# Autodesk Inventor assembly: Double door
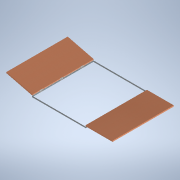
[picture p0: Inventor's stored thumbnail of the model, 180x180]
Saved by Autodesk Inventor 2021 (Build 250183000, 183)
## iProperties
Created: 2021-07-31
Part Number: Double door
Document SubType Name: Assembly
Designer: Shammy Haider
Author: Shammy Haider
## Documents named in this file (4)
- D:\Designing\Autodesk inventor\Wood Door\Double door.iam
- D:\Designing\Autodesk inventor\Wood Door\Frame2.ipt
- D:\Designing\Autodesk inventor\Wood Door\Hinge assembly.iam
- D:\Designing\Autodesk inventor\Wood Door\Door.ipt
## Components (9 placed, 3 different names)
1. Frame2:1 — Mate:1, Mate:2, Mate:3, Mate:4, Mate:5, Mate:6, Mate:7, Mate:8, Mate:9, Mate:10, Mate:11, Mate:12, Mate:13, Mate:14, Mate:15, Mate:16, Mate:17, Mate:18
2. Hinge assembly:1 [sub-assembly] — Mate:1, Mate:2, Mate:3, Mate:20, Mate:23
3. Hinge assembly:2 [sub-assembly] — Mate:13, Mate:16, Mate:17, Mate:21, Mate:22
4. Hinge assembly:3 [sub-assembly] — Mate:14, Mate:15, Mate:18, Mate:19
5. Hinge assembly:4 [sub-assembly] — Mate:10, Mate:11, Mate:12, Mate:26
6. Hinge assembly:5 [sub-assembly] — Mate:7, Mate:8, Mate:9, Mate:25, Mate:27
7. Hinge assembly:6 [sub-assembly] — Mate:4, Mate:5, Mate:6, Mate:24
8. Door:2 — Mate:19, Mate:20, Mate:21, Mate:22, Mate:23
9. Door:3 — Mate:24, Mate:25, Mate:26, Mate:27
## Relationships (27: Mate 27)
- Mate:1: Frame2:1 ↔ Hinge assembly:1
- Mate:2: Frame2:1 ↔ Hinge assembly:1
- Mate:3: Frame2:1 ↔ Hinge assembly:1
- Mate:4: Frame2:1 ↔ Hinge assembly:6
- Mate:5: Frame2:1 ↔ Hinge assembly:6
- Mate:6: Frame2:1 ↔ Hinge assembly:6
- Mate:7: Frame2:1 ↔ Hinge assembly:5
- Mate:8: Frame2:1 ↔ Hinge assembly:5
- Mate:9: Frame2:1 ↔ Hinge assembly:5
- Mate:10: Frame2:1 ↔ Hinge assembly:4
- Mate:11: Frame2:1 ↔ Hinge assembly:4
- Mate:12: Frame2:1 ↔ Hinge assembly:4
- Mate:13: Frame2:1 ↔ Hinge assembly:2
- Mate:14: Frame2:1 ↔ Hinge assembly:3
- Mate:15: Frame2:1 ↔ Hinge assembly:3
- Mate:16: Frame2:1 ↔ Hinge assembly:2
- Mate:17: Frame2:1 ↔ Hinge assembly:2
- Mate:18: Frame2:1 ↔ Hinge assembly:3
- Mate:19: Hinge assembly:3 ↔ Door:2
- Mate:20: Hinge assembly:1 ↔ Door:2
- Mate:21: Hinge assembly:2 ↔ Door:2
- Mate:22: Hinge assembly:2 ↔ Door:2
- Mate:23: Hinge assembly:1 ↔ Door:2
- Mate:24: Hinge assembly:6 ↔ Door:3
- Mate:25: Hinge assembly:5 ↔ Door:3
- Mate:26: Hinge assembly:4 ↔ Door:3
- Mate:27: Hinge assembly:5 ↔ Door:3
